# Autodesk Inventor assembly: Assembly1
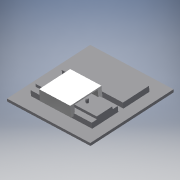
[picture p0: Inventor's stored thumbnail of the model, 180x180]
Saved by Autodesk Inventor 2019.4 (Build 234330000, 330)
## iProperties
Created: 2020-11-10
Part Number: Assembly1
Document SubType Name: Assembly
Designer: caleb
Author: caleb
## Documents named in this file (3)
- C:\Users\cfang\Desktop\CAD\TFPX\glue spreader jig\Assembly1.iam
- C:\Users\cfang\Desktop\CAD\TFPX\glue spreader jig\main body.ipt
- C:\Users\cfang\Desktop\CAD\TFPX\glue spreader jig\Assembly Station with parts.iam
## Components (2 placed, 2 different names)
1. main body:1 — Mate:3, Mate:4, Mate:5
2. Assembly Station with parts:1 [sub-assembly] — Mate:3, Mate:4, Mate:5
## Relationships (3: Mate 3)
- Mate:3: main body:1 ↔ Assembly Station with parts:1
- Mate:4: main body:1 ↔ Assembly Station with parts:1
- Mate:5: main body:1 ↔ Assembly Station with parts:1
